# Autodesk Inventor assembly: złożenie gąsienicy
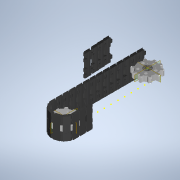
[picture p0: Inventor's stored thumbnail of the model, 180x180]
Saved by Autodesk Inventor 2021 (Build 250183000, 183)
## iProperties
Created: 2021-06-19
Part Number: złożenie gąsienicy
Document SubType Name: Assembly
Designer: Łukasz
Author: Łukasz
## Documents named in this file (6)
- E:\GITHUB_Czołg\Szybki-Czolg-antyRadziecki\złożenie gąsienicy.iam
- E:\GITHUB_Czołg\Szybki-Czolg-antyRadziecki\gąsienica.ipt
- E:\GITHUB_Czołg\Szybki-Czolg-antyRadziecki\koło napędowe.ipt
- E:\GITHUB_Czołg\Szybki-Czolg-antyRadziecki\koło łożyskowane.ipt
- E:\GITHUB_Czołg\Szybki-Czolg-antyRadziecki\dystans łożyska.ipt
- C:\Users\Łukasz\Documents\Inventor\Content Center Files\R2021\en-US\BS 292 (I)\BS 292 Part 1 - 6001 - 12 x 28 x 8.ipt
## Components (30 placed, 5 different names)
1. gąsienica:1 — Rotational:1, Angle:1, Rotational:6, Angle:6
2. gąsienica:2 — Rotational:1, Angle:1, Rotational:2, Angle:2
3. gąsienica:3 — Rotational:5, Angle:5, Rotational:7, Angle:8
4. gąsienica:4 — Rotational:3, Angle:3, Rotational:4, Angle:4, Flush:2
5. gąsienica:5 — Rotational:2, Angle:2, Rotational:3, Angle:3, Mate:1, Flush:1
6. gąsienica:6 — Rotational:6, Angle:6, Rotational:9, Angle:7
7. gąsienica:7 — Rotational:4, Angle:4, Rotational:5, Angle:5
8. gąsienica:8 — Rotational:7, Rotational:8, Angle:8, Angle:9
9. gąsienica:9 — Rotational:8, Angle:9
10. gąsienica:10 — Rotational:9, Angle:7, Rotational:10, Angle:10
11. koło napędowe:1 — Mate:1, Flush:1, Flush:2, Flush:3, Mate:2, Flush:4
12. koło łożyskowane:1 — Flush:3, Mate:2, Insert:1, Insert:2, Insert:3, Flush:4
13. dystans łożyska:1 — Insert:1
14. BS 292: Part 1 (I) (Metric) 6001 - 12 x 28 x 8:1 — Insert:2
15. BS 292: Part 1 (I) (Metric) 6001 - 12 x 28 x 8:2 — Insert:3
16. gąsienica:11 — Rotational:10, Rotational:11, Angle:10, Angle:11
17. gąsienica:12 — Rotational:11, Angle:11, Rotational:12, Angle:12
18. gąsienica:13 — Rotational:13, Rotational:14, Angle:13, Angle:14
19. gąsienica:14 — Rotational:14, Angle:14, Rotational:15, Angle:15
20. gąsienica:15 — Rotational:15, Rotational:16, Angle:15, Angle:16
21. gąsienica:16 — Rotational:12, Rotational:13, Angle:12, Angle:13
22. gąsienica:17 — Rotational:16, Angle:16, Rotational:17, Angle:17
23. gąsienica:18 — Rotational:17, Rotational:18, Angle:17, Angle:18
24. gąsienica:19 — Rotational:18, Angle:18, Rotational:19, Angle:19
25. gąsienica:20 — Rotational:19, Rotational:20, Angle:19, Angle:20
26. gąsienica:21 — Rotational:20, Angle:20
27. gąsienica:22
28. gąsienica:23
29. gąsienica:24
30. gąsienica:25
## Relationships (49: RevoluteJoint 20, Angle 20, Flush 4, Insert 3, Mate 2)
- Rotational:1 [RevoluteJoint]: gąsienica:1 ↔ gąsienica:2
- Angle:1 (-36 deg): gąsienica:1 ↔ gąsienica:2
- Rotational:2 [RevoluteJoint]: gąsienica:2 ↔ gąsienica:5
- Angle:2 (36 deg): gąsienica:2 ↔ gąsienica:5
- Rotational:3 [RevoluteJoint]: gąsienica:4 ↔ gąsienica:5
- Angle:3 (36 deg): gąsienica:4 ↔ gąsienica:5
- Rotational:4 [RevoluteJoint]: gąsienica:4 ↔ gąsienica:7
- Angle:4 (36 deg): gąsienica:4 ↔ gąsienica:7
- Rotational:5 [RevoluteJoint]: gąsienica:3 ↔ gąsienica:7
- Angle:5 (36 deg): gąsienica:3 ↔ gąsienica:7
- Rotational:6 [RevoluteJoint]: gąsienica:1 ↔ gąsienica:6
- Angle:6 (0 deg): gąsienica:1 ↔ gąsienica:6
- Rotational:7 [RevoluteJoint]: gąsienica:3 ↔ gąsienica:8
- Rotational:8 [RevoluteJoint]: gąsienica:8 ↔ gąsienica:9
- Rotational:9 [RevoluteJoint]: gąsienica:6 ↔ gąsienica:10
- Angle:7 (0 deg): gąsienica:6 ↔ gąsienica:10
- Angle:8 (0 deg): gąsienica:3 ↔ gąsienica:8
- Angle:9 (0 deg): gąsienica:8 ↔ gąsienica:9
- Mate:1 (1 mm): gąsienica:5 ↔ koło napędowe:1
- Flush:1: gąsienica:5 ↔ koło napędowe:1
- Flush:2: gąsienica:4 ↔ koło napędowe:1
- Flush:3: koło napędowe:1 ↔ koło łożyskowane:1
- Mate:2 (-310 mm): koło napędowe:1 ↔ koło łożyskowane:1
- Insert:1 (8 mm): koło łożyskowane:1 ↔ dystans łożyska:1
- Insert:2: koło łożyskowane:1 ↔ BS 292: Part 1 (I) (Metric) 6001 - 12 x 28 x 8:1
- Insert:3: koło łożyskowane:1 ↔ BS 292: Part 1 (I) (Metric) 6001 - 12 x 28 x 8:2
- Rotational:10 [RevoluteJoint]: gąsienica:10 ↔ gąsienica:11
- Rotational:11 [RevoluteJoint]: gąsienica:11 ↔ gąsienica:12
- Angle:10 (0 deg): gąsienica:10 ↔ gąsienica:11
- Angle:11 (0 deg): gąsienica:11 ↔ gąsienica:12
- Rotational:12 [RevoluteJoint]: gąsienica:12 ↔ gąsienica:16
- Rotational:13 [RevoluteJoint]: gąsienica:13 ↔ gąsienica:16
- Rotational:14 [RevoluteJoint]: gąsienica:13 ↔ gąsienica:14
- Angle:12 (0 deg): gąsienica:12 ↔ gąsienica:16
- Angle:13 (0 deg): gąsienica:13 ↔ gąsienica:16
- Angle:14 (0 deg): gąsienica:13 ↔ gąsienica:14
- Rotational:15 [RevoluteJoint]: gąsienica:14 ↔ gąsienica:15
- Rotational:16 [RevoluteJoint]: gąsienica:15 ↔ gąsienica:17
- Angle:15 (0 deg): gąsienica:14 ↔ gąsienica:15
- Angle:16 (0 deg): gąsienica:15 ↔ gąsienica:17
- Rotational:17 [RevoluteJoint]: gąsienica:17 ↔ gąsienica:18
- Rotational:18 [RevoluteJoint]: gąsienica:18 ↔ gąsienica:19
- Angle:17 (0 deg): gąsienica:17 ↔ gąsienica:18
- Angle:18 (0 deg): gąsienica:18 ↔ gąsienica:19
- Rotational:19 [RevoluteJoint]: gąsienica:19 ↔ gąsienica:20
- Rotational:20 [RevoluteJoint]: gąsienica:20 ↔ gąsienica:21
- Angle:19 (0 deg): gąsienica:19 ↔ gąsienica:20
- Angle:20 (0 deg): gąsienica:20 ↔ gąsienica:21
- Flush:4: koło napędowe:1 ↔ koło łożyskowane:1
